# Autodesk Inventor assembly: flash assy
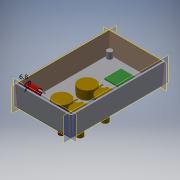
[picture p0: Inventor's stored thumbnail of the model, 180x180]
Saved by Autodesk Inventor 2018 (Build 220112000, 112)
## iProperties
Created: 2017-12-11
Part Number: flash assy
Document SubType Name: Assembly
Designer: caleb
Author: caleb
## Documents named in this file (6)
- C:\cygwin64\home\caleb\wifi-flash-trigger\simple-flash-trigger\inventor\flash assy.iam
- C:\cygwin64\home\caleb\wifi-flash-trigger\simple-flash-trigger\inventor\box_bottom.ipt
- C:\cygwin64\home\caleb\wifi-flash-trigger\simple-flash-trigger\inventor\potentiometer.ipt
- C:\cygwin64\home\caleb\wifi-flash-trigger\simple-flash-trigger\inventor\arduino.ipt
- C:\cygwin64\home\caleb\wifi-flash-trigger\simple-flash-trigger\inventor\switch.ipt
- C:\cygwin64\home\caleb\wifi-flash-trigger\simple-flash-trigger\inventor\headphone jack.ipt
## Components (8 placed, 5 different names)
1. box_bottom:1 — Mate:1, Mate:2, Mate:3, Mate:4, Mate:6, Flush:8, Mate:7
2. potentiometer:1 — Mate:1, Flush:1, Flush:6, Flush:7
3. potentiometer:2 — Mate:2, Flush:1, Flush:2
4. potentiometer:3 — Flush:2, Flush:3, Flush:4, Flush:5
5. potentiometer:4 — Flush:3, Mate:3, Flush:4, Flush:5, Flush:6, Flush:7
6. arduino:1 — Mate:4, Mate:5
7. switch:1 — Mate:6
8. headphone jack:1 — Flush:8, Mate:7
## Relationships (15: Flush 8, Mate 7)
- Mate:1: box_bottom:1 ↔ potentiometer:1
- Mate:2: box_bottom:1 ↔ potentiometer:2
- Flush:1: potentiometer:1 ↔ potentiometer:2
- Flush:2: potentiometer:2 ↔ potentiometer:3
- Flush:3: potentiometer:3 ↔ potentiometer:4
- Mate:3: box_bottom:1 ↔ potentiometer:4
- Flush:4: potentiometer:3 ↔ potentiometer:4
- Mate:4: box_bottom:1 ↔ arduino:1
- Mate:5: arduino:1
- Flush:5 (19.05 mm): potentiometer:3 ↔ potentiometer:4
- Flush:6: potentiometer:1 ↔ potentiometer:4
- Flush:7 (26.67 mm): potentiometer:1 ↔ potentiometer:4
- Mate:6: box_bottom:1 ↔ switch:1
- Flush:8 (-3 mm): box_bottom:1 ↔ headphone jack:1
- Mate:7: box_bottom:1 ↔ headphone jack:1
